# Autodesk Inventor assembly: Carriage Assembly V1
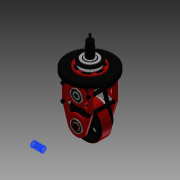
[picture p0: Inventor's stored thumbnail of the model, 180x180]
Saved by Autodesk Inventor 2013 (Build 170138000, 138)
## iProperties
Created: 2013-04-01
Part Number: Carriage Assembly V1
Document SubType Name: Assembly
Designer: mvarma
Author: mvarma
## Documents named in this file (34)
- C:\Users\mvarma\Desktop\Swerve Gearbox\Swerve Gearbox V1\Carriage Assembly V1.iam
- C:\Users\mvarma\Desktop\Swerve Gearbox\Swerve Gearbox V1\Carriage Plate - Bolt Head Side.ipt
- C:\Users\mvarma\Desktop\Swerve Gearbox\Swerve Gearbox V1\Carriage Plate - Gear Mount.ipt
- C:\Users\mvarma\Desktop\Swerve Gearbox\Swerve Gearbox V1\Carriage Plate - Pem Nut Side.ipt
- C:\Users\mvarma\Desktop\Swerve Gearbox\Swerve Gearbox V1\Imported Components\10-32 Thread Pem Nut.ipt
- C:\Users\mvarma\Desktop\Swerve Gearbox\Swerve Gearbox V1\Imported Components\Socket Head Cap Screw 10-32 Thread .500 Length.ipt
- C:\Users\mvarma\Desktop\Swerve Gearbox\Swerve Gearbox V1\Carriage Standoff - 2.125 Long.ipt
- C:\Users\mvarma\Desktop\Swerve Gearbox\Swerve Gearbox V1\Imported Components\Socket Head Cap Screw 10-32 Thread 2.500 Length.ipt
- C:\Users\mvarma\Desktop\Swerve Gearbox\Swerve Gearbox V1\Imported Components\84t Tooth Gear .500 Hex Bore.ipt
- C:\Users\mvarma\Desktop\Swerve Gearbox\Swerve Gearbox V1\Imported Components\FR8-2RS.ipt
- C:\Users\mvarma\Desktop\Swerve Gearbox\Swerve Gearbox V1\Carriage Shaft - Lower.ipt
- C:\Users\mvarma\Desktop\Swerve Gearbox\Swerve Gearbox V1\Carriage Shaft - Upper.ipt
- C:\Users\mvarma\Desktop\Swerve Gearbox\Swerve Gearbox V1\Wheel - Tread.ipt
- C:\Users\mvarma\Desktop\Swerve Gearbox\Swerve Gearbox V1\Wheel - Rim.ipt
- C:\Users\mvarma\Desktop\Swerve Gearbox\Swerve Gearbox V1\Carriage Spacer - Wheel.ipt
- C:\Users\mvarma\Desktop\Swerve Gearbox\Swerve Gearbox V1\Imported Components\Socket Head Cap Screw 8-32 Thread .750 Length.ipt
- C:\Users\mvarma\Desktop\Swerve Gearbox\Swerve Gearbox V1\Carriage Plate - Gear Cover.ipt
- C:\Users\mvarma\Desktop\Swerve Gearbox\Swerve Gearbox V1\Imported Components\FR6-2RS.ipt
- C:\Users\mvarma\Desktop\Swerve Gearbox\Swerve Gearbox V1\Imported Components\20t Tooth Gear .375 Hex Bore Miter 1.125 Mounting Distance  - Upper Carriage Gear.ipt
- C:\Users\mvarma\Desktop\Swerve Gearbox\Swerve Gearbox V1\Imported Components\20t Tooth Gear .375 Hex Bore Miter 1.125 Mounting Distance  - Carriage Input Gear.ipt
- C:\Users\mvarma\Desktop\Swerve Gearbox\Swerve Gearbox V1\Carriage Shaft - Input.ipt
- C:\Users\mvarma\Desktop\Swerve Gearbox\Swerve Gearbox V1\Carriage Spacer - Upper.ipt
- C:\Users\mvarma\Desktop\Swerve Gearbox\Swerve Gearbox V1\Imported Components\Slotted Spring Pin - .125 OD .750 Long.ipt
- C:\Users\mvarma\Desktop\Swerve Gearbox\Swerve Gearbox V1\Imported Components\64t Tooth Pulley .500 Hex Bore 3mm GT2.ipt
- C:\Users\mvarma\Desktop\Swerve Gearbox\Swerve Gearbox V1\Imported Components\24t Tooth Pulley .375 Hex Bore 3mm GT2.ipt
- C:\Users\mvarma\Desktop\Swerve Gearbox\Swerve Gearbox V1\Carriage Spacer - Input.ipt
- C:\Users\mvarma\Desktop\Swerve Gearbox\Swerve Gearbox V1\Imported Components\Black-Finish Steel External Retaining Ring .500 Shaft Diameter.ipt
- C:\Users\mvarma\Desktop\Swerve Gearbox\Swerve Gearbox V1\Imported Components\FR10-2RS.ipt
- C:\Users\mvarma\Desktop\Swerve Gearbox\Swerve Gearbox V1\Imported Components\Bronze Thrust Bearing.125 Thick .500 Shaft Diameter 1.000 OD.ipt
- C:\Users\mvarma\Desktop\Swerve Gearbox\Swerve Gearbox V1\Thrust Bearing Assembly Bushing 1.125 Shaft Diameter.ipt
- C:\Users\mvarma\Desktop\Swerve Gearbox\Swerve Gearbox V1\Imported Components\Thrust Washer .032 Thick 1.125 Shaft Diameter.ipt
- C:\Users\mvarma\Desktop\Swerve Gearbox\Swerve Gearbox V1\Imported Components\Thrust Needle-Roller Bearing 1.125 Shaft Diameter.ipt
- C:\Users\mvarma\Desktop\Swerve Gearbox\Swerve Gearbox V1\Carriage Spacer - Thrust Bearing.ipt
- C:\Users\mvarma\Desktop\Swerve Gearbox\Swerve Gearbox V1\Timming Belt - 165 mm.ipt
## Components (55 placed, 33 different names)
1. Black-Finish Steel External Retaining Ring .500 Shaft Diameter:1 — Mate:170, Mate:172
2. Black-Finish Steel External Retaining Ring .500 Shaft Diameter:2 — Mate:171, Mate:173
3. Slotted Spring Pin - .125 OD .750 Long:1 — Mate:166, Mate:167, Mate:168
4. 10-32 Thread Pem Nut:1 — Mate:79, Mate:85
5. 10-32 Thread Pem Nut:2 — Mate:80, Mate:84
6. 10-32 Thread Pem Nut:3 — Mate:78, Mate:86
7. 10-32 Thread Pem Nut:4 — Mate:77, Mate:83
8. Carriage Plate - Bolt Head Side:1 — Mate:1, Mate:2, Mate:3, Mate:7, Mate:8, Mate:9, Mate:10, Mate:11, Mate:12, Mate:37, Mate:38, Mate:41, Mate:42, Mate:43, Mate:44, Mate:45, Mate:46, Mate:48, Mate:49, Mate:50, Mate:51, Mate:52, Mate:53, Mate:55, Mate:56, Mate:61, Mate:64, Mate:68, Mate:69, Mate:72, Mate:74, Mate:75, Mate:105, Mate:107, Mate:109, Angle:1, Mate:135, Mate:171
9. Carriage Plate - Gear Mount:1 — Mate:1, Mate:2, Mate:3, Mate:4, Mate:5, Mate:6, Mate:57, Mate:58, Mate:59, Mate:87, Mate:88, Mate:89, Mate:90, Mate:91, Mate:92, Mate:93, Mate:94, Mate:95, Mate:96, Mate:114, Angle:2, Mate:157, Mate:158, Mate:159, Mate:169, Mate:175, Mate:176, Mate:180
10. Carriage Plate - Pem Nut Side:1 — Mate:4, Mate:5, Mate:6, Mate:13, Mate:14, Mate:15, Mate:16, Mate:17, Mate:18, Mate:62, Mate:67, Mate:77, Mate:78, Mate:79, Mate:80, Mate:83, Mate:84, Mate:85, Mate:86, Mate:106, Mate:108, Mate:140, Angle:3, Mate:170, Mate:187, Mate:188
11. Carriage Plate - Gear Cover:1 — Mate:95, Mate:96, Mate:97, Mate:181
12. Carriage Shaft - Lower:1 — Flush:2, Mate:69, Mate:73, Mate:130, Mate:143, Mate:172, Mate:173
13. Carriage Shaft - Upper:1 — Mate:68, Flush:3, Mate:110, Mate:111, Mate:136, Mate:144, Mate:145, Flush:5
14. Carriage Shaft - Input:1 — Mate:168, Mate:169, Mate:184, Mate:185
15. Carriage Spacer - Thrust Bearing:1 — Mate:182, Mate:186
16. Carriage Spacer - Input:1 — Mate:159, Flush:9
17. Carriage Spacer - Upper:1 — Mate:135, Mate:136, Mate:146
18. Carriage Spacer - Wheel:1 — Mate:75, Mate:76, Mate:130
19. Carriage Standoff - 2.125 Long:1 — Mate:37, Mate:38
20. Carriage Standoff - 2.125 Long:2 — Mate:41, Mate:42
21. Carriage Standoff - 2.125 Long:4 — Mate:45, Mate:46
22. Carriage Standoff - 2.125 Long:5 — Mate:43, Mate:44
23. Wheel - Tread:1 — Mate:70, Mate:71, Tangent:5
24. Wheel - Rim:1 — Mate:70, Mate:71, Mate:72, Mate:73, Mate:74, Mate:76, Mate:142
25. Socket Head Cap Screw 8-32 Thread .750 Length:1 — Mate:88, Mate:92
26. Socket Head Cap Screw 8-32 Thread .750 Length:2 — Mate:89, Mate:93
27. Socket Head Cap Screw 8-32 Thread .750 Length:3 — Mate:87, Mate:91
28. Socket Head Cap Screw 8-32 Thread .750 Length:4 — Mate:90, Mate:94
29. Socket Head Cap Screw 10-32 Thread 2.500 Length:1 — Mate:48, Mate:53
30. Socket Head Cap Screw 10-32 Thread 2.500 Length:2 — Mate:51, Mate:56
31. Socket Head Cap Screw 10-32 Thread 2.500 Length:3 — Mate:49, Mate:55
32. Socket Head Cap Screw 10-32 Thread 2.500 Length:4 — Mate:50, Mate:52
33. Socket Head Cap Screw 10-32 Thread .500 Length:1 — Mate:7, Mate:8
34. Socket Head Cap Screw 10-32 Thread .500 Length:2 — Mate:15, Mate:17
35. Socket Head Cap Screw 10-32 Thread .500 Length:3 — Mate:16, Mate:18
36. Socket Head Cap Screw 10-32 Thread .500 Length:4 — Mate:13, Mate:14
37. Socket Head Cap Screw 10-32 Thread .500 Length:5 — Mate:9, Mate:10
38. Socket Head Cap Screw 10-32 Thread .500 Length:6 — Mate:11, Mate:12
39. FR6-2RS:1 — Mate:105, Mate:107, Flush:3
40. FR6-2RS:2 — Mate:106, Mate:108
41. FR8-2RS:4 — Mate:157, Mate:158, Mate:174
42. FR8-2RS:1 — Mate:61, Mate:64, Flush:2
43. FR8-2RS:3 — Mate:62, Mate:67
44. Bronze Thrust Bearing.125 Thick .500 Shaft Diameter 1.000 OD:1 — Mate:174, Mate:175
45. FR10-2RS:1 — Mate:176, Mate:182, Mate:186
46. Thrust Needle-Roller Bearing 1.125 Shaft Diameter:1 — Mate:177, Tangent:6
47. Thrust Washer .032 Thick 1.125 Shaft Diameter:1 — Mate:179, Flush:7, Tangent:6, Mate:181
48. Thrust Washer .032 Thick 1.125 Shaft Diameter:2 — Mate:178, Flush:8
49. Thrust Bearing Assembly Bushing 1.125 Shaft Diameter:1 — Mate:177, Mate:178, Mate:179, Flush:7, Flush:8, Mate:180
50. Timming Belt - 165 mm:1 — Mate:187, Mate:188, Mate:189
51. 20t Tooth Gear .375 Hex Bore Miter 1.125 Mounting Distance  - Upper Carriage Gear:1 — Mate:109, Mate:110, Mate:111, Angle:1, Mate:146, Mate:165
52. 20t Tooth Gear .375 Hex Bore Miter 1.125 Mounting Distance  - Carriage Input Gear:1 — Mate:114, Angle:2, Mate:165, Mate:166, Mate:167
53. 84t Tooth Gear .500 Hex Bore:1 — Mate:57, Mate:58, Mate:59, Mate:97, Flush:9
54. 24t Tooth Pulley .375 Hex Bore 3mm GT2:1 — Mate:144, Mate:145, Flush:5, Mate:189
55. 64t Tooth Pulley .500 Hex Bore 3mm GT2:1 — Mate:140, Mate:142, Mate:143, Angle:3
## Relationships (125: Mate 113, Flush 6, Angle 4, Tangent 2)
- Mate:1: Carriage Plate - Bolt Head Side:1 ↔ Carriage Plate - Gear Mount:1
- Mate:2: Carriage Plate - Bolt Head Side:1 ↔ Carriage Plate - Gear Mount:1
- Mate:3: Carriage Plate - Bolt Head Side:1 ↔ Carriage Plate - Gear Mount:1
- Mate:4: Carriage Plate - Gear Mount:1 ↔ Carriage Plate - Pem Nut Side:1
- Mate:5: Carriage Plate - Gear Mount:1 ↔ Carriage Plate - Pem Nut Side:1
- Mate:6: Carriage Plate - Gear Mount:1 ↔ Carriage Plate - Pem Nut Side:1
- Mate:7: Carriage Plate - Bolt Head Side:1 ↔ Socket Head Cap Screw 10-32 Thread .500 Length:1
- Mate:8: Carriage Plate - Bolt Head Side:1 ↔ Socket Head Cap Screw 10-32 Thread .500 Length:1
- Mate:9: Carriage Plate - Bolt Head Side:1 ↔ Socket Head Cap Screw 10-32 Thread .500 Length:5
- Mate:10: Carriage Plate - Bolt Head Side:1 ↔ Socket Head Cap Screw 10-32 Thread .500 Length:5
- Mate:11: Carriage Plate - Bolt Head Side:1 ↔ Socket Head Cap Screw 10-32 Thread .500 Length:6
- Mate:12: Carriage Plate - Bolt Head Side:1 ↔ Socket Head Cap Screw 10-32 Thread .500 Length:6
- Mate:13: Carriage Plate - Pem Nut Side:1 ↔ Socket Head Cap Screw 10-32 Thread .500 Length:4
- Mate:14: Carriage Plate - Pem Nut Side:1 ↔ Socket Head Cap Screw 10-32 Thread .500 Length:4
- Mate:15: Carriage Plate - Pem Nut Side:1 ↔ Socket Head Cap Screw 10-32 Thread .500 Length:2
- Mate:16: Carriage Plate - Pem Nut Side:1 ↔ Socket Head Cap Screw 10-32 Thread .500 Length:3
- Mate:17: Carriage Plate - Pem Nut Side:1 ↔ Socket Head Cap Screw 10-32 Thread .500 Length:2
- Mate:18: Carriage Plate - Pem Nut Side:1 ↔ Socket Head Cap Screw 10-32 Thread .500 Length:3
- Mate:37: Carriage Plate - Bolt Head Side:1 ↔ Carriage Standoff - 2.125 Long:1
- Mate:38: Carriage Plate - Bolt Head Side:1 ↔ Carriage Standoff - 2.125 Long:1
- Mate:41: Carriage Plate - Bolt Head Side:1 ↔ Carriage Standoff - 2.125 Long:2
- Mate:42: Carriage Plate - Bolt Head Side:1 ↔ Carriage Standoff - 2.125 Long:2
- Mate:43: Carriage Plate - Bolt Head Side:1 ↔ Carriage Standoff - 2.125 Long:5
- Mate:44: Carriage Plate - Bolt Head Side:1 ↔ Carriage Standoff - 2.125 Long:5
- Mate:45: Carriage Plate - Bolt Head Side:1 ↔ Carriage Standoff - 2.125 Long:4
- Mate:46: Carriage Plate - Bolt Head Side:1 ↔ Carriage Standoff - 2.125 Long:4
- Mate:48: Carriage Plate - Bolt Head Side:1 ↔ Socket Head Cap Screw 10-32 Thread 2.500 Length:1
- Mate:49: Carriage Plate - Bolt Head Side:1 ↔ Socket Head Cap Screw 10-32 Thread 2.500 Length:3
- Mate:50: Carriage Plate - Bolt Head Side:1 ↔ Socket Head Cap Screw 10-32 Thread 2.500 Length:4
- Mate:51: Carriage Plate - Bolt Head Side:1 ↔ Socket Head Cap Screw 10-32 Thread 2.500 Length:2
- Mate:52: Carriage Plate - Bolt Head Side:1 ↔ Socket Head Cap Screw 10-32 Thread 2.500 Length:4
- Mate:53: Carriage Plate - Bolt Head Side:1 ↔ Socket Head Cap Screw 10-32 Thread 2.500 Length:1
- Mate:55: Carriage Plate - Bolt Head Side:1 ↔ Socket Head Cap Screw 10-32 Thread 2.500 Length:3
- Mate:56: Carriage Plate - Bolt Head Side:1 ↔ Socket Head Cap Screw 10-32 Thread 2.500 Length:2
- Mate:57: Carriage Plate - Gear Mount:1 ↔ 84t Tooth Gear .500 Hex Bore:1
- Mate:58: Carriage Plate - Gear Mount:1 ↔ 84t Tooth Gear .500 Hex Bore:1
- Mate:59: Carriage Plate - Gear Mount:1 ↔ 84t Tooth Gear .500 Hex Bore:1
- Mate:61: Carriage Plate - Bolt Head Side:1 ↔ FR8-2RS:1
- Mate:62: Carriage Plate - Pem Nut Side:1 ↔ FR8-2RS:3
- Mate:64: Carriage Plate - Bolt Head Side:1 ↔ FR8-2RS:1
- Mate:67: Carriage Plate - Pem Nut Side:1 ↔ FR8-2RS:3
- Flush:2: Carriage Shaft - Lower:1 ↔ FR8-2RS:1
- Mate:68: Carriage Plate - Bolt Head Side:1 ↔ Carriage Shaft - Upper:1
- Mate:69: Carriage Plate - Bolt Head Side:1 ↔ Carriage Shaft - Lower:1
- Mate:70: Wheel - Tread:1 ↔ Wheel - Rim:1
- Mate:71: Wheel - Tread:1 ↔ Wheel - Rim:1
- Mate:72: Carriage Plate - Bolt Head Side:1 ↔ Wheel - Rim:1
- Mate:73: Carriage Shaft - Lower:1 ↔ Wheel - Rim:1
- Mate:74 (14.2875 mm): Carriage Plate - Bolt Head Side:1 ↔ Wheel - Rim:1
- Mate:75: Carriage Plate - Bolt Head Side:1 ↔ Carriage Spacer - Wheel:1
- Mate:76: Carriage Spacer - Wheel:1 ↔ Wheel - Rim:1
- Mate:77: 10-32 Thread Pem Nut:4 ↔ Carriage Plate - Pem Nut Side:1
- Mate:78: 10-32 Thread Pem Nut:3 ↔ Carriage Plate - Pem Nut Side:1
- Mate:79: 10-32 Thread Pem Nut:1 ↔ Carriage Plate - Pem Nut Side:1
- Mate:80: 10-32 Thread Pem Nut:2 ↔ Carriage Plate - Pem Nut Side:1
- Mate:83: 10-32 Thread Pem Nut:4 ↔ Carriage Plate - Pem Nut Side:1
- Mate:84: 10-32 Thread Pem Nut:2 ↔ Carriage Plate - Pem Nut Side:1
- Mate:85: 10-32 Thread Pem Nut:1 ↔ Carriage Plate - Pem Nut Side:1
- Mate:86: 10-32 Thread Pem Nut:3 ↔ Carriage Plate - Pem Nut Side:1
- Mate:87: Carriage Plate - Gear Mount:1 ↔ Socket Head Cap Screw 8-32 Thread .750 Length:3
- Mate:88: Carriage Plate - Gear Mount:1 ↔ Socket Head Cap Screw 8-32 Thread .750 Length:1
- Mate:89: Carriage Plate - Gear Mount:1 ↔ Socket Head Cap Screw 8-32 Thread .750 Length:2
- Mate:90: Carriage Plate - Gear Mount:1 ↔ Socket Head Cap Screw 8-32 Thread .750 Length:4
- Mate:91: Carriage Plate - Gear Mount:1 ↔ Socket Head Cap Screw 8-32 Thread .750 Length:3
- Mate:92: Carriage Plate - Gear Mount:1 ↔ Socket Head Cap Screw 8-32 Thread .750 Length:1
- Mate:93: Carriage Plate - Gear Mount:1 ↔ Socket Head Cap Screw 8-32 Thread .750 Length:2
- Mate:94: Carriage Plate - Gear Mount:1 ↔ Socket Head Cap Screw 8-32 Thread .750 Length:4
- Mate:95: Carriage Plate - Gear Mount:1 ↔ Carriage Plate - Gear Cover:1
- Mate:96: Carriage Plate - Gear Mount:1 ↔ Carriage Plate - Gear Cover:1
- Mate:97: Carriage Plate - Gear Cover:1 ↔ 84t Tooth Gear .500 Hex Bore:1
- Mate:105: Carriage Plate - Bolt Head Side:1 ↔ FR6-2RS:1
- Mate:106: Carriage Plate - Pem Nut Side:1 ↔ FR6-2RS:2
- Mate:107: Carriage Plate - Bolt Head Side:1 ↔ FR6-2RS:1
- Mate:108: Carriage Plate - Pem Nut Side:1 ↔ FR6-2RS:2
- Flush:3: Carriage Shaft - Upper:1 ↔ FR6-2RS:1
- Mate:109: Carriage Plate - Bolt Head Side:1 ↔ 20t Tooth Gear .375 Hex Bore Miter 1.125 Mounting Distance  - Upper Carriage Gear:1
- Mate:110: Carriage Shaft - Upper:1 ↔ 20t Tooth Gear .375 Hex Bore Miter 1.125 Mounting Distance  - Upper Carriage Gear:1
- Mate:111: Carriage Shaft - Upper:1 ↔ 20t Tooth Gear .375 Hex Bore Miter 1.125 Mounting Distance  - Upper Carriage Gear:1
- Mate:114: Carriage Plate - Gear Mount:1 ↔ 20t Tooth Gear .375 Hex Bore Miter 1.125 Mounting Distance  - Carriage Input Gear:1
- Angle:1 (0 deg): Carriage Plate - Bolt Head Side:1 ↔ 20t Tooth Gear .375 Hex Bore Miter 1.125 Mounting Distance  - Upper Carriage Gear:1
- Angle:2 (9 deg): Carriage Plate - Gear Mount:1 ↔ 20t Tooth Gear .375 Hex Bore Miter 1.125 Mounting Distance  - Carriage Input Gear:1
- Mate:130: Carriage Shaft - Lower:1 ↔ Carriage Spacer - Wheel:1
- Mate:135: Carriage Plate - Bolt Head Side:1 ↔ Carriage Spacer - Upper:1
- Mate:136: Carriage Shaft - Upper:1 ↔ Carriage Spacer - Upper:1
- Mate:140: Carriage Plate - Pem Nut Side:1 ↔ 64t Tooth Pulley .500 Hex Bore 3mm GT2:1
- Mate:142: Wheel - Rim:1 ↔ 64t Tooth Pulley .500 Hex Bore 3mm GT2:1
- Mate:143: Carriage Shaft - Lower:1 ↔ 64t Tooth Pulley .500 Hex Bore 3mm GT2:1
- Mate:144: Carriage Shaft - Upper:1 ↔ 24t Tooth Pulley .375 Hex Bore 3mm GT2:1
- Mate:145: Carriage Shaft - Upper:1 ↔ 24t Tooth Pulley .375 Hex Bore 3mm GT2:1
- Flush:5: Carriage Shaft - Upper:1 ↔ 24t Tooth Pulley .375 Hex Bore 3mm GT2:1
- Mate:146: Carriage Spacer - Upper:1 ↔ 20t Tooth Gear .375 Hex Bore Miter 1.125 Mounting Distance  - Upper Carriage Gear:1
- Angle:3 (0 deg): Carriage Plate - Pem Nut Side:1 ↔ 64t Tooth Pulley .500 Hex Bore 3mm GT2:1
- Mate:157: Carriage Plate - Gear Mount:1 ↔ FR8-2RS:4
- Mate:158: Carriage Plate - Gear Mount:1 ↔ FR8-2RS:4
- Mate:159: Carriage Plate - Gear Mount:1 ↔ Carriage Spacer - Input:1
- Mate:165: 20t Tooth Gear .375 Hex Bore Miter 1.125 Mounting Distance  - Upper Carriage Gear:1 ↔ 20t Tooth Gear .375 Hex Bore Miter 1.125 Mounting Distance  - Carriage Input Gear:1
- Mate:166: Slotted Spring Pin - .125 OD .750 Long:1 ↔ 20t Tooth Gear .375 Hex Bore Miter 1.125 Mounting Distance  - Carriage Input Gear:1
- Mate:167: Slotted Spring Pin - .125 OD .750 Long:1 ↔ 20t Tooth Gear .375 Hex Bore Miter 1.125 Mounting Distance  - Carriage Input Gear:1
- Mate:168: Slotted Spring Pin - .125 OD .750 Long:1 ↔ Carriage Shaft - Input:1
- Mate:169: Carriage Plate - Gear Mount:1 ↔ Carriage Shaft - Input:1
- Mate:170: Black-Finish Steel External Retaining Ring .500 Shaft Diameter:1 ↔ Carriage Plate - Pem Nut Side:1
- Mate:171: Black-Finish Steel External Retaining Ring .500 Shaft Diameter:2 ↔ Carriage Plate - Bolt Head Side:1
- Mate:172 (0.0508 mm): Black-Finish Steel External Retaining Ring .500 Shaft Diameter:1 ↔ Carriage Shaft - Lower:1
- Mate:173 (0.0508 mm): Black-Finish Steel External Retaining Ring .500 Shaft Diameter:2 ↔ Carriage Shaft - Lower:1
- Angle:4 (0 deg)
- Tangent:5: Wheel - Tread:1
- Mate:174: FR8-2RS:4 ↔ Bronze Thrust Bearing.125 Thick .500 Shaft Diameter 1.000 OD:1
- Mate:175: Carriage Plate - Gear Mount:1 ↔ Bronze Thrust Bearing.125 Thick .500 Shaft Diameter 1.000 OD:1
- Mate:176: Carriage Plate - Gear Mount:1 ↔ FR10-2RS:1
- Mate:177: Thrust Needle-Roller Bearing 1.125 Shaft Diameter:1 ↔ Thrust Bearing Assembly Bushing 1.125 Shaft Diameter:1
- Mate:178: Thrust Washer .032 Thick 1.125 Shaft Diameter:2 ↔ Thrust Bearing Assembly Bushing 1.125 Shaft Diameter:1
- Mate:179: Thrust Washer .032 Thick 1.125 Shaft Diameter:1 ↔ Thrust Bearing Assembly Bushing 1.125 Shaft Diameter:1
- Flush:7: Thrust Washer .032 Thick 1.125 Shaft Diameter:1 ↔ Thrust Bearing Assembly Bushing 1.125 Shaft Diameter:1
- Flush:8: Thrust Washer .032 Thick 1.125 Shaft Diameter:2 ↔ Thrust Bearing Assembly Bushing 1.125 Shaft Diameter:1
- Tangent:6: Thrust Needle-Roller Bearing 1.125 Shaft Diameter:1 ↔ Thrust Washer .032 Thick 1.125 Shaft Diameter:1
- Mate:180: Carriage Plate - Gear Mount:1 ↔ Thrust Bearing Assembly Bushing 1.125 Shaft Diameter:1
- Mate:181: Carriage Plate - Gear Cover:1 ↔ Thrust Washer .032 Thick 1.125 Shaft Diameter:1
- Flush:9: Carriage Spacer - Input:1 ↔ 84t Tooth Gear .500 Hex Bore:1
- Mate:182: Carriage Spacer - Thrust Bearing:1 ↔ FR10-2RS:1
- Mate:184: Carriage Shaft - Input:1
- Mate:185: Carriage Shaft - Input:1
- Mate:186: Carriage Spacer - Thrust Bearing:1 ↔ FR10-2RS:1
- Mate:187: Carriage Plate - Pem Nut Side:1 ↔ Timming Belt - 165 mm:1
- Mate:188: Carriage Plate - Pem Nut Side:1 ↔ Timming Belt - 165 mm:1
- Mate:189: Timming Belt - 165 mm:1 ↔ 24t Tooth Pulley .375 Hex Bore 3mm GT2:1
## Named parameters: x = 0 deg
